# Autodesk Inventor assembly: Assembly1
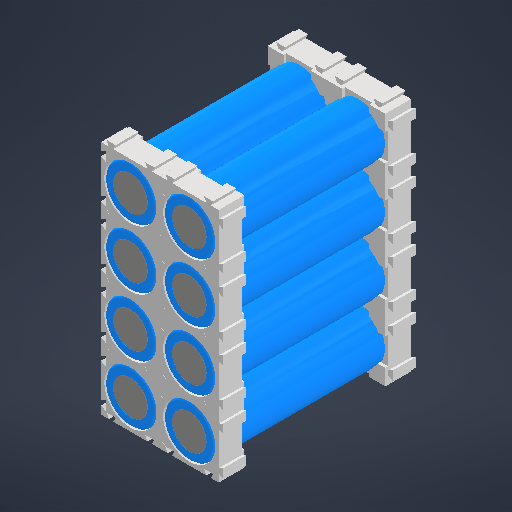
[picture p0: Inventor's stored thumbnail of the model, 512x512]
Saved by Autodesk Inventor 2026.1 (Build 301233000, 233)
## iProperties
Created: 2026-03-05
Part Number: Assembly1
Document SubType Name: Assembly
Designer: ghon0
Author: ghon0
## Documents named in this file (4)
- D:\momen\Eng.-ASU\Senior1\MCT Sys design\design\battery pack\Assembly1.iam
- D:\momen\Eng.-ASU\Senior1\MCT Sys design\design\battery pack\Battery 18650.ipt
- D:\momen\Eng.-ASU\Senior1\MCT Sys design\design\battery pack\Battery Holder.ipt
- D:\momen\Eng.-ASU\Senior1\MCT Sys design\design\battery pack\Battery Holder_MIR.ipt
## Components (24 placed, 3 different names)
1. Battery 18650:3 — Mate:6, Flush:6
2. Battery Holder:1 — Mate:1, Flush:1, Mate:2, Flush:2, Flush:3, Mate:3, Mate:5
3. Battery 18650:2 — Mate:5, Flush:5, Flush:6
4. Battery Holder:3 — Flush:2, Flush:3, Mate:3, Mate:6
5. Battery Holder_MIR:3 — Mate:9, Flush:8, Flush:9
6. Battery Holder_MIR:1 — Mate:7, Flush:7, Mate:8, Mate:9, Flush:8, Flush:9
7. Battery 18650:5
8. Battery Holder:5
9. Battery 18650:6
10. Battery Holder:6
11. Battery Holder_MIR:5
12. Battery Holder_MIR:6
13. Battery Holder_MIR:2 — Mate:7, Flush:7, Mate:8
14. Battery 18650:1 — Mate:4, Flush:4, Flush:5
15. Battery Holder:2 — Mate:1, Flush:1, Mate:2, Mate:4, Flush:4
16. Battery Holder_MIR:4
17. Battery 18650:4
18. Battery Holder:4
19. Battery Holder_MIR:7
20. Battery 18650:7
21. Battery Holder:7
22. Battery Holder_MIR:8
23. Battery 18650:8
24. Battery Holder:8
## Component patterns: (2 elements, first: Battery 18650:3 + Battery Holder:1 + Battery 18650:2 + Battery Holder:3 + Battery Holder_MIR:3 + Battery Holder_MIR:1), (2 elements, first: Battery Holder_MIR:2 + Battery 18650:1 + Battery Holder:2), Component Pattern 2:2 (2 elements)
## Relationships (18: Mate 9, Flush 9)
- Mate:1: Battery Holder:1 ↔ Battery Holder:2
- Flush:1: Battery Holder:1 ↔ Battery Holder:2
- Mate:2: Battery Holder:1 ↔ Battery Holder:2
- Flush:2: Battery Holder:1 ↔ Battery Holder:3
- Flush:3: Battery Holder:1 ↔ Battery Holder:3
- Mate:3: Battery Holder:1 ↔ Battery Holder:3
- Mate:4: Battery 18650:1 ↔ Battery Holder:2
- Flush:4: Battery 18650:1 ↔ Battery Holder:2
- Mate:5: Battery Holder:1 ↔ Battery 18650:2
- Mate:6: Battery 18650:3 ↔ Battery Holder:3
- Flush:5: Battery 18650:2 ↔ Battery 18650:1
- Flush:6: Battery 18650:3 ↔ Battery 18650:2
- Mate:7: Battery Holder_MIR:1 ↔ Battery Holder_MIR:2
- Flush:7: Battery Holder_MIR:1 ↔ Battery Holder_MIR:2
- Mate:8: Battery Holder_MIR:1 ↔ Battery Holder_MIR:2
- Mate:9: Battery Holder_MIR:3 ↔ Battery Holder_MIR:1
- Flush:8: Battery Holder_MIR:3 ↔ Battery Holder_MIR:1
- Flush:9: Battery Holder_MIR:3 ↔ Battery Holder_MIR:1
